# Autodesk Inventor assembly: Omni Robot
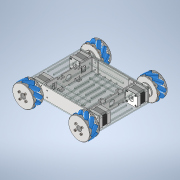
[picture p0: Inventor's stored thumbnail of the model, 180x180]
Saved by Autodesk Inventor 2021 (Build 250183000, 183)
## iProperties
Created: 2022-05-03
Part Number: Omni Robot
Document SubType Name: Assembly
Designer: 21155308
Author: 21155308
## Documents named in this file (7)
- U:\Projeto\Omni Robot.iam
- U:\Projeto\Base.ipt
- U:\Projeto\chapa lateral.ipt
- U:\Projeto\MINEBEA 05701607 stepper motor.ipt
- U:\Projeto\chapa lentral.ipt
- U:\Projeto\roda direita\Mecanum Wheel Assembly Right-r4.iam
- U:\Projeto\roda esquerda\Mecanum Wheel Assembly Left-r4.iam
## Components (14 placed, 6 different names)
1. Base:1 — Coincidente:1, Alinhado:1, Alinhado:3, Coincidente:5, Coincidente:19, Coincidente:21
2. Base:2 — Coincidente:2, Alinhado:2, Coincidente:3, Alinhado:4, Alinhado:5
3. chapa lateral:1 — Coincidente:1, Coincidente:2, Alinhado:1, Alinhado:2, Alinhado:3, Coincidente:3, Coincidente:6, Coincidente:7, Coincidente:8, Coincidente:12, Coincidente:13, Coincidente:14, Coincidente:18, Coincidente:20, Alinhado:7, Coincidente:23, Coincidente:25
4. chapa lateral:2 — Coincidente:5, Alinhado:4, Alinhado:5, Coincidente:9, Coincidente:10, Coincidente:11, Coincidente:15, Coincidente:16, Coincidente:17, Alinhado:6, Coincidente:27, Coincidente:29
5. MINEBEA 05701607 stepper motor:1 — Coincidente:9, Coincidente:10, Coincidente:11, Coincidente:28
6. MINEBEA 05701607 stepper motor:2 — Coincidente:6, Coincidente:7, Coincidente:8, Coincidente:24
7. MINEBEA 05701607 stepper motor:3 — Coincidente:15, Coincidente:16, Coincidente:17, Coincidente:26
8. MINEBEA 05701607 stepper motor:4 — Coincidente:12, Coincidente:13, Coincidente:14, Coincidente:22
9. chapa lentral:1 — Coincidente:18, Coincidente:19, Alinhado:7
10. chapa lentral:2 — Coincidente:20, Coincidente:21, Alinhado:6
11. Mecanum Wheel Assembly Right-r4:1 [sub-assembly] — Coincidente:22, Coincidente:23
12. Mecanum Wheel Assembly Right-r4:2 [sub-assembly] — Coincidente:28, Coincidente:29
13. Mecanum Wheel Assembly Left-r4:1 [sub-assembly] — Coincidente:24, Coincidente:25
14. Mecanum Wheel Assembly Left-r4:2 [sub-assembly] — Coincidente:26, Coincidente:27
## Relationships (35: Mate 28, Flush 7)
- Coincidente:1 [Mate]: Base:1 ↔ chapa lateral:1
- Coincidente:2 [Mate]: Base:2 ↔ chapa lateral:1
- Alinhado:1 [Flush]: Base:1 ↔ chapa lateral:1
- Alinhado:2 [Flush]: Base:2 ↔ chapa lateral:1
- Alinhado:3 [Flush]: Base:1 ↔ chapa lateral:1
- Coincidente:3 [Mate]: Base:2 ↔ chapa lateral:1
- Coincidente:5 [Mate]: Base:1 ↔ chapa lateral:2
- Alinhado:4 [Flush]: Base:2 ↔ chapa lateral:2
- Alinhado:5 [Flush]: Base:2 ↔ chapa lateral:2
- Coincidente:6 [Mate]: chapa lateral:1 ↔ MINEBEA 05701607 stepper motor:2
- Coincidente:7 [Mate]: chapa lateral:1 ↔ MINEBEA 05701607 stepper motor:2
- Coincidente:8 [Mate]: chapa lateral:1 ↔ MINEBEA 05701607 stepper motor:2
- Coincidente:9 [Mate]: chapa lateral:2 ↔ MINEBEA 05701607 stepper motor:1
- Coincidente:10 [Mate]: chapa lateral:2 ↔ MINEBEA 05701607 stepper motor:1
- Coincidente:11 [Mate]: chapa lateral:2 ↔ MINEBEA 05701607 stepper motor:1
- Coincidente:12 [Mate]: chapa lateral:1 ↔ MINEBEA 05701607 stepper motor:4
- Coincidente:13 [Mate]: chapa lateral:1 ↔ MINEBEA 05701607 stepper motor:4
- Coincidente:14 [Mate]: chapa lateral:1 ↔ MINEBEA 05701607 stepper motor:4
- Coincidente:15 [Mate]: chapa lateral:2 ↔ MINEBEA 05701607 stepper motor:3
- Coincidente:16 [Mate]: chapa lateral:2 ↔ MINEBEA 05701607 stepper motor:3
- Coincidente:17 [Mate]: chapa lateral:2 ↔ MINEBEA 05701607 stepper motor:3
- Coincidente:18 [Mate]: chapa lateral:1 ↔ chapa lentral:1
- Coincidente:19 [Mate]: Base:1 ↔ chapa lentral:1
- Coincidente:20 [Mate]: chapa lateral:1 ↔ chapa lentral:2
- Coincidente:21 [Mate]: Base:1 ↔ chapa lentral:2
- Alinhado:6 [Flush] (42 mm): chapa lateral:2 ↔ chapa lentral:2
- Alinhado:7 [Flush] (42 mm): chapa lateral:1 ↔ chapa lentral:1
- Coincidente:22 [Mate]: MINEBEA 05701607 stepper motor:4 ↔ Mecanum Wheel Assembly Right-r4:1
- Coincidente:23 [Mate] (10 mm): chapa lateral:1 ↔ Mecanum Wheel Assembly Right-r4:1
- Coincidente:24 [Mate]: MINEBEA 05701607 stepper motor:2 ↔ Mecanum Wheel Assembly Left-r4:1
- Coincidente:25 [Mate] (10 mm): chapa lateral:1 ↔ Mecanum Wheel Assembly Left-r4:1
- Coincidente:26 [Mate]: MINEBEA 05701607 stepper motor:3 ↔ Mecanum Wheel Assembly Left-r4:2
- Coincidente:27 [Mate] (10 mm): chapa lateral:2 ↔ Mecanum Wheel Assembly Left-r4:2
- Coincidente:28 [Mate]: MINEBEA 05701607 stepper motor:1 ↔ Mecanum Wheel Assembly Right-r4:2
- Coincidente:29 [Mate] (10 mm): chapa lateral:2 ↔ Mecanum Wheel Assembly Right-r4:2
